# Autodesk Inventor assembly: FH01-10SS
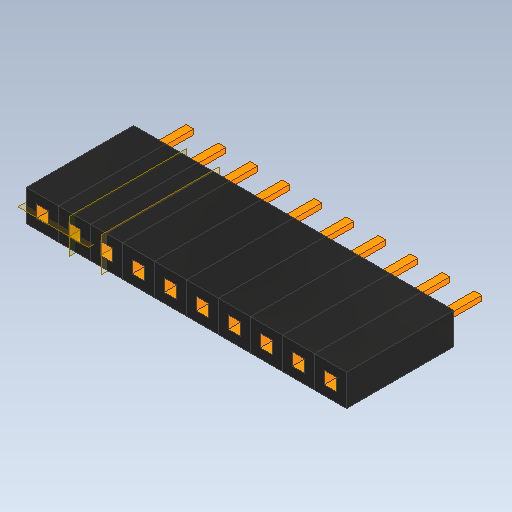
[picture p0: Inventor's stored thumbnail of the model, 512x512]
Saved by Autodesk Inventor 2020.2 (Build 242310000, 310)
## iProperties
Created: 2020-01-01
Part Number: FH01-10SS
Description: STEP AP214
Document SubType Name: Assembly
Designer: Tarsoly
Preprocessor: Spatial InterOp 3D
Title: FH01-10SS.stp
Revision Number: NONE
## Documents named in this file (3)
- D:\Users\Tarsoly\Dokumentumok\BME\Dipterv\3d\pins\socket\10x1\FH01-10SS.iam
- D:\Users\Tarsoly\Dokumentumok\BME\Dipterv\3d\pins\socket\10x1\Part1.ipt
- D:\Users\Tarsoly\Dokumentumok\BME\Dipterv\3d\pins\socket\10x1\Part3.ipt
## Components (20 placed, 4 different names)
1. Part1 — Symmetry:1, Symmetry:2
2. Part3
3. Cnt1 — Symmetry:2, Symmetry:3
4. Cnt2
5. Part1:1 — Symmetry:1
6. Part3:1
7. Part1:2 — Symmetry:3
8. Part3:2
9. Part1:3
10. Part3:3
11. Part1:4
12. Part3:4
13. Part1:5
14. Part3:5
15. Part1:6
16. Part3:6
17. Part1:7
18. Part3:7
19. Part1:8
20. Part3:8
## Relationships (7: Mate 4, Symmetry 3)
- Symmetry:1: Part1 ↔ Part1:1
- Symmetry:2: Part1 ↔ Cnt1
- Mate:1
- Mate:2
- Symmetry:3: Cnt1 ↔ Part1:2
- Mate:3
- Mate:4
